# Autodesk Inventor assembly: robot_simplified
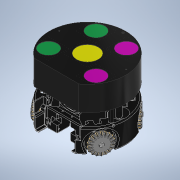
[picture p0: Inventor's stored thumbnail of the model, 180x180]
Saved by Autodesk Inventor 2021 (Build 250183000, 183)
## iProperties
Created: 2022-09-21
Part Number: robot_simplified
Document SubType Name: Assembly
Designer: victo
Author: victo
## Documents named in this file (11)
- C:\Users\victo\Documents\MATLAB\CAD\Inventor\robot_simplified.iam
- C:\Users\victo\Documents\MATLAB\CAD\Inventor\2021\Base_RoboCIn.ipt
- C:\Users\victo\Documents\MATLAB\CAD\Inventor\2021\SupportFirstToSecond.ipt
- C:\Users\victo\Documents\MATLAB\CAD\Inventor\2021\plate_sec_floor.ipt
- C:\Users\victo\Documents\MATLAB\CAD\Inventor\2021\SupportSecondToCoverNew.ipt
- C:\Users\victo\Documents\MATLAB\CAD\Inventor\2021\CoverNew.ipt
- C:\Users\victo\Documents\MATLAB\CAD\Inventor\2021\tag_green.ipt
- C:\Users\victo\Documents\MATLAB\CAD\Inventor\2021\tag_magenta.ipt
- C:\Users\victo\Documents\MATLAB\CAD\Inventor\2021\tag_yellow.ipt
- C:\Users\victo\Documents\MATLAB\CAD\Inventor\sec_floor\tampa_nut.ipt
- C:\Users\victo\Documents\MATLAB\CAD\Inventor\first_floor\Wheel\RoboCinWheel_simplified.iam
## Components (19 placed, 10 different names)
1. Base_RoboCIn:1 — Mate:1, Mate:2, Mate:3, Mate:4
2. SupportFirstToSecond:1
3. SupportFirstToSecond:2
4. SupportFirstToSecond:3
5. SupportFirstToSecond:4
6. plate_sec_floor:1
7. SupportSecondToCoverNew:1
8. SupportSecondToCoverNew:2
9. CoverNew:1
10. tag_green:1
11. tag_green:2
12. tag_magenta:1
13. tag_magenta:2
14. tag_yellow:1
15. tampa_nut:1
16. RoboCinWheel_simplified:1 [sub-assembly] — Mate:1
17. RoboCinWheel_simplified:2 [sub-assembly] — Mate:2
18. RoboCinWheel_simplified:3 [sub-assembly] — Mate:3
19. RoboCinWheel_simplified:4 [sub-assembly] — Mate:4
## Relationships (4: Mate 4)
- Mate:1: Base_RoboCIn:1 ↔ RoboCinWheel_simplified:1
- Mate:2: Base_RoboCIn:1 ↔ RoboCinWheel_simplified:2
- Mate:3: Base_RoboCIn:1 ↔ RoboCinWheel_simplified:3
- Mate:4: Base_RoboCIn:1 ↔ RoboCinWheel_simplified:4
